# Autodesk Inventor assembly: Assembly2
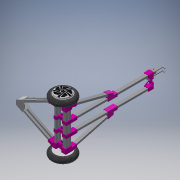
[picture p0: Inventor's stored thumbnail of the model, 180x180]
Saved by Autodesk Inventor 2018.3 (Build 223284000, 284)
## iProperties
Created: 2020-09-11
Part Number: Assembly2
Document SubType Name: Assembly
Designer: chris
Author: chris
## Documents named in this file (12)
- C:\Users\chris\Documents\Z Desktop\Lina-Chris Proj\DriveTrain_Assembly.iam
- C:\Users\chris\Documents\Z Desktop\Lina-Chris Proj\Motor_BLDC_Hoverboard_Wheel.ipt
- C:\Users\chris\Documents\Z Desktop\Lina-Chris Proj\PL_rod_single.ipt
- C:\Users\chris\Documents\Z Desktop\Lina-Chris Proj\Left_front_Chasis_v2.ipt
- C:\Users\chris\Documents\Z Desktop\Lina-Chris Proj\Right_front_Chasis_v2.ipt
- C:\Users\chris\Documents\Z Desktop\Lina-Chris Proj\PL_rod_double.ipt
- C:\Users\chris\Documents\Z Desktop\Lina-Chris Proj\mid_front_Chasis.ipt
- C:\Users\chris\Documents\Z Desktop\Lina-Chris Proj\upper_joints.ipt
- C:\Users\chris\Documents\Z Desktop\Lina-Chris Proj\backwheel_Mount.ipt
- C:\Users\chris\Documents\Z Desktop\Lina-Chris Proj\tablet_arm_joint.ipt
- C:\Users\chris\Documents\Z Desktop\Lina-Chris Proj\Tablet_joint_Holder.ipt
- C:\Users\chris\Documents\Z Desktop\Lina-Chris Proj\tab_clips.ipt
## Components (27 placed, 11 different names)
1. Motor_BLDC_Hoverboard_Wheel:1 — Rigid:10
2. Motor_BLDC_Hoverboard_Wheel:2 — Rigid:1
3. PL_rod_single:1 — Rigid:6
4. PL_rod_single:2 — Rigid:7
5. PL_rod_single:3 — Rigid:8
6. PL_rod_single:4 — Rigid:5
7. Left_front_Chasis_v2:1 — Rigid:1, Rigid:5, Rigid:6, Rigid:7, Rigid:8, Rigid:15, Rigid:17, Rigid:21
8. Right_front_Chasis_v2:1 — Rigid:10, Rigid:12, Rigid:13, Rigid:14, Rigid:16, Rigid:20
9. PL_rod_single:5 — Rigid:13, Rigid:24
10. PL_rod_single:6 — Rigid:12
11. PL_rod_double:1 — Rigid:15
12. PL_rod_double:2 — Rigid:18, Rigid:22
13. PL_rod_double:3 — Rigid:19, Rigid:23
14. PL_rod_double:4 — Rigid:20
15. PL_rod_double:5 — Rigid:14
16. PL_rod_double:6 — Rigid:21
17. mid_front_Chasis:1 — Rigid:16, Rigid:19
18. mid_front_Chasis:2 — Rigid:17, Rigid:18
19. upper_joints:1 — Rigid:22, Rigid:25
20. upper_joints:2 — Rigid:23, Rigid:26
21. backwheel_Mount:1 — Rigid:24
22. PL_rod_double:7 — Rigid:25
23. PL_rod_double:8 — Rigid:26, Rigid:27
24. tablet_arm_joint:1 — Rigid:28, Rotational:1, Rotational:2
25. Tablet_joint_Holder:1 — Rigid:27, Rigid:28
26. tab_clips:1 — Rotational:1
27. tab_clips:2 — Rotational:2
## Relationships (25: WeldJoint 23, RevoluteJoint 2)
- Rigid:1 [WeldJoint]: Motor_BLDC_Hoverboard_Wheel:2 ↔ Left_front_Chasis_v2:1
- Rigid:5 [WeldJoint]: PL_rod_single:4 ↔ Left_front_Chasis_v2:1
- Rigid:6 [WeldJoint]: PL_rod_single:1 ↔ Left_front_Chasis_v2:1
- Rigid:7 [WeldJoint]: PL_rod_single:2 ↔ Left_front_Chasis_v2:1
- Rigid:8 [WeldJoint]: PL_rod_single:3 ↔ Left_front_Chasis_v2:1
- Rigid:10 [WeldJoint]: Motor_BLDC_Hoverboard_Wheel:1 ↔ Right_front_Chasis_v2:1
- Rigid:12 [WeldJoint]: Right_front_Chasis_v2:1 ↔ PL_rod_single:6
- Rigid:13 [WeldJoint]: Right_front_Chasis_v2:1 ↔ PL_rod_single:5
- Rigid:14 [WeldJoint]: Right_front_Chasis_v2:1 ↔ PL_rod_double:5
- Rigid:15 [WeldJoint]: Left_front_Chasis_v2:1 ↔ PL_rod_double:1
- Rigid:16 [WeldJoint] (73 mm): Right_front_Chasis_v2:1 ↔ mid_front_Chasis:1
- Rigid:17 [WeldJoint] (73 mm): Left_front_Chasis_v2:1 ↔ mid_front_Chasis:2
- Rigid:18 [WeldJoint]: PL_rod_double:2 ↔ mid_front_Chasis:2
- Rigid:19 [WeldJoint]: PL_rod_double:3 ↔ mid_front_Chasis:1
- Rigid:20 [WeldJoint]: Right_front_Chasis_v2:1 ↔ PL_rod_double:4
- Rigid:21 [WeldJoint]: Left_front_Chasis_v2:1 ↔ PL_rod_double:6
- Rigid:22 [WeldJoint]: PL_rod_double:2 ↔ upper_joints:1
- Rigid:23 [WeldJoint]: PL_rod_double:3 ↔ upper_joints:2
- Rigid:24 [WeldJoint]: PL_rod_single:5 ↔ backwheel_Mount:1
- Rigid:25 [WeldJoint]: upper_joints:1 ↔ PL_rod_double:7
- Rigid:26 [WeldJoint]: upper_joints:2 ↔ PL_rod_double:8
- Rigid:27 [WeldJoint]: PL_rod_double:8 ↔ Tablet_joint_Holder:1
- Rigid:28 [WeldJoint]: tablet_arm_joint:1 ↔ Tablet_joint_Holder:1
- Rotational:1 [RevoluteJoint]: tablet_arm_joint:1 ↔ tab_clips:1
- Rotational:2 [RevoluteJoint]: tablet_arm_joint:1 ↔ tab_clips:2
